# Autodesk Inventor assembly: Robot
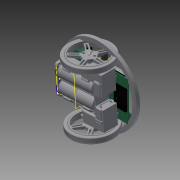
[picture p0: Inventor's stored thumbnail of the model, 180x180]
Saved by Autodesk Inventor 2014 (Build 180170000, 170)
## iProperties
Created: 2013-06-25
Part Number: Robot
Document SubType Name: Assembly
Designer: Felix
Author: Felix
## Documents named in this file (5)
- C:\Users\Felix\Desktop\Robot\Robot.iam
- C:\Users\Felix\Desktop\Robot\Pololu_gear_motor_1_180\gear_motor.iam
- C:\Users\Felix\Desktop\Robot\Pololu_Wheel_6mm\Wheel.iam
- C:\Users\Felix\Desktop\Robot\battery_holder\holder_with_batteries.iam
- C:\Users\Felix\Desktop\Robot\RaspberryPi\RaspberryPi_with_frame.iam
## Components (6 placed, 4 different names)
1. gear_motor:1 [sub-assembly] — Passend:1, Passend:5, Passend:6, Passend:7, Fluchtend:3, Fluchtend:4, Passend:8, Passend:10, Passend:11
2. gear_motor:2 [sub-assembly] — Passend:1, Passend:2, Passend:3, Passend:4, Fluchtend:3, Passend:9
3. Wheel:1 [sub-assembly] — Passend:5, Passend:6, Passend:7
4. Wheel:2 [sub-assembly] — Passend:2, Passend:3, Passend:4
5. holder_with_batteries:1 [sub-assembly] — Fluchtend:4, Passend:8, Passend:9, Passend:10
6. RaspberryPi_with_frame:1 [sub-assembly] — Passend:11
## Relationships (13: Mate 11, Flush 2)
- Passend:1 [Mate]: gear_motor:1 ↔ gear_motor:2
- Passend:2 [Mate]: gear_motor:2 ↔ Wheel:2
- Passend:3 [Mate]: gear_motor:2 ↔ Wheel:2
- Passend:4 [Mate]: gear_motor:2 ↔ Wheel:2
- Passend:5 [Mate]: gear_motor:1 ↔ Wheel:1
- Passend:6 [Mate]: gear_motor:1 ↔ Wheel:1
- Passend:7 [Mate]: gear_motor:1 ↔ Wheel:1
- Fluchtend:3 [Flush]: gear_motor:1 ↔ gear_motor:2
- Fluchtend:4 [Flush]: gear_motor:1 ↔ holder_with_batteries:1
- Passend:8 [Mate]: gear_motor:1 ↔ holder_with_batteries:1
- Passend:9 [Mate]: gear_motor:2 ↔ holder_with_batteries:1
- Passend:10 [Mate]: gear_motor:1 ↔ holder_with_batteries:1
- Passend:11 [Mate]: gear_motor:1 ↔ RaspberryPi_with_frame:1
